# Autodesk Inventor assembly: lens-clamp-hsi
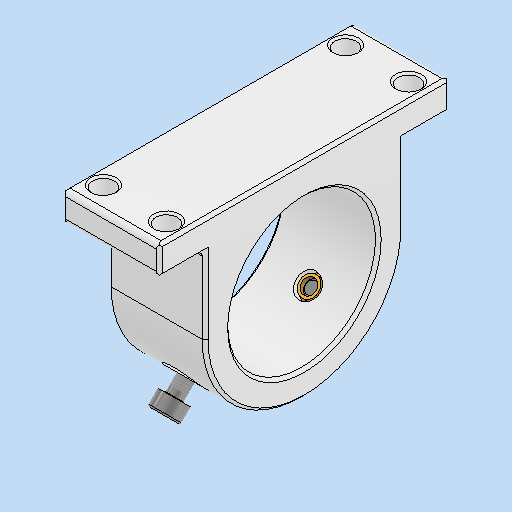
[picture p0: Inventor's stored thumbnail of the model, 512x512]
Saved by Autodesk Inventor 2025 (Build 290162000, 162)
## iProperties
Created: 2025-06-06
Part Number: lens-clamp-hsi
Document SubType Name: Assembly
Designer: kuzmin
Author: kuzmin
## Documents named in this file (4)
- C:\Users\queez\Dropbox\Drawings\PIHTI\LIBS\lens-clamp-hsi.iam
- C:\Users\queez\Dropbox\Drawings\PIHTI\LIBS\lens-clamp.ipt
- C:\Users\queez\Dropbox\Drawings\PIHTI\ContentCenter\Fastners\brass-insert-m3x5.ipt
- C:\Users\queez\Dropbox\Drawings\PIHTI\ContentCenter\Fastners\M3x8-SHCS.ipt
## Components (5 placed, 3 different names)
1. lens-clamp:1
2. brass-insert-m3x5:1 — Mate:1
3. brass-insert-m3x5:2 — Mate:2
4. SS ISO 4762 M3 x 8:1 — Mate:1
5. SS ISO 4762 M3 x 8:2 — Mate:2
## Relationships (4: WeldJoint 2, Mate 2)
- [WeldJoint]: lens-clamp:1 ↔ brass-insert-m3x5:1
- [WeldJoint]: lens-clamp:1 ↔ brass-insert-m3x5:2
- Mate:1: brass-insert-m3x5:1 ↔ SS ISO 4762 M3 x 8:1
- Mate:2: brass-insert-m3x5:2 ↔ SS ISO 4762 M3 x 8:2
